# Autodesk Inventor assembly: mount3
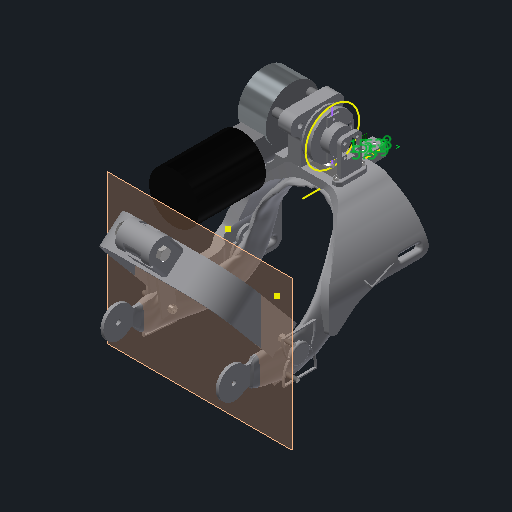
[picture p0: Inventor's stored thumbnail of the model, 512x512]
Saved by Autodesk Inventor 2025.2 (Build 292293000, 293)
## iProperties
Created: 2025-02-11
Part Number: mount3
Document SubType Name: Assembly
Designer: Alex
Author: Alex
## Documents named in this file (14)
- C:\Shared\alex-bartella-schoolwork\4tb6\4TB6-repo\CAD_Model\thigh_mount_2\thighmount_assembly_2.1.iam
- C:\Shared\alex-bartella-schoolwork\4tb6\4TB6-repo\CAD_Model\thigh_mount_2\thigh.ipt
- C:\Shared\alex-bartella-schoolwork\4tb6\4TB6-repo\CAD_Model\thigh_mount_2\thighmount2.1.ipt
- C:\Shared\alex-bartella-schoolwork\4tb6\4TB6-repo\CAD_Model\thigh_mount_2\motor.ipt
- C:\Shared\alex-bartella-schoolwork\4tb6\4TB6-repo\CAD_Model\thigh_mount_2\spool_temp.ipt
- C:\Shared\alex-bartella-schoolwork\4tb6\4TB6-repo\CAD_Model\thigh_mount_2\magnetholder.ipt
- C:\Shared\alex-bartella-schoolwork\4tb6\4TB6-repo\CAD_Model\thigh_mount_2\imu_house_assembly.iam
- C:\Shared\alex-bartella-schoolwork\4tb6\4TB6-repo\CAD_Model\thigh_mount_2\as5600mount_2.ipt
- C:\Shared\alex-bartella-schoolwork\4tb6\4TB6-repo\CAD_Model\thigh_mount_2\pulley_bracket_assem.iam
- C:\Shared\alex-bartella-schoolwork\4tb6\4TB6-repo\CAD_Model\thigh_mount_2\brace_tabs.ipt
- C:\Shared\alex-bartella-schoolwork\4tb6\4TB6-repo\CAD_Model\thigh_mount_2\brace_tabs_half.ipt
- C:\Shared\alex-bartella-schoolwork\4tb6\4TB6-repo\CAD_Model\thigh_mount_2\short_L_bracket.ipt
- C:\Shared\alex-bartella-schoolwork\4tb6\4TB6-repo\CAD_Model\thigh_mount_2\fasteners\ANSI B18.6.7M - M6x1 x 13(6).ipt
- C:\Users\turbo\Documents\Inventor\Content Center Files\R2025\en-US\AS 1420\AS 1420 - 1973 - M3 x 6.ipt
## Components (19 placed, 13 different names)
1. thigh:1 — Mate:1, Mate:2, Flush:1, Mate:28, Mate:29, Mate:30, Mate:31, Mate:32, Mate:33
2. thighmount2.1:1 — Flush:4, Mate:3, Mate:4, Mate:5, Angle:7, Angle:2, Mate:21, Mate:22, Mate:27, Mate:34, Angle:8, Flush:5, Flush:6
3. motor:1 — Mate:3, Mate:4, Mate:5, Mate:7, Mate:23
4. spool_temp:1 — Mate:7, Mate:9, Mate:10, Mate:11, Mate:23
5. magnetholder:1 — Mate:9, Mate:10, Mate:11, Mate:18, Mate:25, Mate:26
6. imu_house_assembly:1 [sub-assembly] — Mate:34, Angle:8, Flush:5, Insert:5
7. as5600mount_2:1 — Mate:18, Mate:25, Mate:26, Mate:27, Insert:3, Insert:4
8. pulley_bracket_assem:1 [sub-assembly] — Angle:7, Angle:2, Mate:21, Mate:22
9. brace_tabs:1 — Mate:28, Mate:29
10. brace_tabs:2 — Mate:30, Mate:31
11. brace_tabs_half:1 — Mate:32
12. brace_tabs_half:2 — Mate:33
13. brace_tabs_half:3
14. short_L_bracket:1 — Flush:6, Insert:1, Insert:2
15. Square Recessed Pan Head Machine Screw - Type III - Metric M6x1 x 13:1 — Insert:1
16. Square Recessed Pan Head Machine Screw - Type III - Metric M6x1 x 13:2 — Insert:2
17. AS 1420 - Metric M3 x 6:1 — Insert:3
18. AS 1420 - Metric M3 x 6:2 — Insert:4
19. AS 1420 - Metric M3 x 6:3 — Insert:5
## Relationships (36: Mate 23, Flush 5, Insert 5, Angle 3)
- Mate:1: thigh:1
- Mate:2: thigh:1
- Flush:1: thigh:1
- Flush:3 (-15 mm)
- Flush:4: thighmount2.1:1
- Mate:3: thighmount2.1:1 ↔ motor:1
- Mate:4: thighmount2.1:1 ↔ motor:1
- Mate:5: thighmount2.1:1 ↔ motor:1
- Mate:7: motor:1 ↔ spool_temp:1
- Mate:9: spool_temp:1 ↔ magnetholder:1
- Mate:10: spool_temp:1 ↔ magnetholder:1
- Mate:11: spool_temp:1 ↔ magnetholder:1
- Mate:18: magnetholder:1 ↔ as5600mount_2:1
- Angle:7 (0 deg): thighmount2.1:1 ↔ pulley_bracket_assem:1
- Angle:2 (-40 deg): thighmount2.1:1 ↔ pulley_bracket_assem:1
- Mate:21 (-30 mm): thighmount2.1:1 ↔ pulley_bracket_assem:1
- Mate:22 (-40 mm): thighmount2.1:1 ↔ pulley_bracket_assem:1
- Mate:23: motor:1 ↔ spool_temp:1
- Mate:25: magnetholder:1 ↔ as5600mount_2:1
- Mate:26 (8 mm): magnetholder:1 ↔ as5600mount_2:1
- Mate:27: thighmount2.1:1 ↔ as5600mount_2:1
- Mate:28: thigh:1 ↔ brace_tabs:1
- Mate:29: thigh:1 ↔ brace_tabs:1
- Mate:30: thigh:1 ↔ brace_tabs:2
- Mate:31: thigh:1 ↔ brace_tabs:2
- Mate:32: thigh:1 ↔ brace_tabs_half:1
- Mate:33 (2 mm): thigh:1 ↔ brace_tabs_half:2
- Mate:34: thighmount2.1:1 ↔ imu_house_assembly:1
- Angle:8 (90 deg): thighmount2.1:1 ↔ imu_house_assembly:1
- Flush:5: thighmount2.1:1 ↔ imu_house_assembly:1
- Flush:6: thighmount2.1:1 ↔ short_L_bracket:1
- Insert:1: short_L_bracket:1 ↔ Square Recessed Pan Head Machine Screw - Type III - Metric M6x1 x 13:1
- Insert:2: short_L_bracket:1 ↔ Square Recessed Pan Head Machine Screw - Type III - Metric M6x1 x 13:2
- Insert:3: as5600mount_2:1 ↔ AS 1420 - Metric M3 x 6:1
- Insert:4: as5600mount_2:1 ↔ AS 1420 - Metric M3 x 6:2
- Insert:5: imu_house_assembly:1 ↔ AS 1420 - Metric M3 x 6:3
